# Autodesk Inventor assembly: The Real Chassis
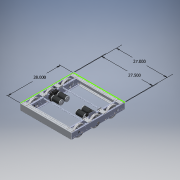
[picture p0: Inventor's stored thumbnail of the model, 180x180]
Saved by Autodesk Inventor 2018 (Build 220112000, 112)
## iProperties
Created: 2015-12-07
Part Number: The Real Chassis
Description: STEP AP214
Document SubType Name: Assembly
Designer: 20dbrownell
Sending System: SolidWorks 2014
Preprocessor: SwSTEP 2.0
Title: AM14U3 Square REV1-1.STEP
Revision Number: ANY
## Documents named in this file (3)
- C:\Users\20dbrownell\Documents\GitHub\RobotDesigns2018\The Real Chassis.iam
- C:\Users\20dbrownell\Downloads\AM14U3 Square Half.iam
- H:\Robotics\am-0255+2.5inch+CIM+Motor.ipt
## Components (10 placed, 3 different names)
1. AM14U3 Square Half_1 [sub-assembly] — Mate:1, Mate:2, Mate:5, Mate:6, Mate:9, Mate:10, Mate:14, Mate:16
2. AM14U3 Square Half_2 [sub-assembly] — Mate:3, Mate:4, Mate:7, Mate:8, Mate:11, Mate:12, Mate:13, Mate:15
3. am-0255+2.5inch+CIM+Motor:1 — Mate:4, Mate:7
4. am-0255+2.5inch+CIM+Motor:2 — Mate:3, Mate:8
5. am-0255+2.5inch+CIM+Motor:3 — Mate:2, Mate:6
6. am-0255+2.5inch+CIM+Motor:4 — Mate:1, Mate:5
7. am-0255+2.5inch+CIM+Motor:5 — Mate:10, Mate:16
8. am-0255+2.5inch+CIM+Motor:6 — Mate:11, Mate:15
9. am-0255+2.5inch+CIM+Motor:7 — Mate:12, Mate:13
10. am-0255+2.5inch+CIM+Motor:8 — Mate:9, Mate:14
## Relationships (16: Mate 16)
- Mate:1: AM14U3 Square Half_1 ↔ am-0255+2.5inch+CIM+Motor:4
- Mate:2: AM14U3 Square Half_1 ↔ am-0255+2.5inch+CIM+Motor:3
- Mate:3: AM14U3 Square Half_2 ↔ am-0255+2.5inch+CIM+Motor:2
- Mate:4: AM14U3 Square Half_2 ↔ am-0255+2.5inch+CIM+Motor:1
- Mate:5: AM14U3 Square Half_1 ↔ am-0255+2.5inch+CIM+Motor:4
- Mate:6: AM14U3 Square Half_1 ↔ am-0255+2.5inch+CIM+Motor:3
- Mate:7: AM14U3 Square Half_2 ↔ am-0255+2.5inch+CIM+Motor:1
- Mate:8: AM14U3 Square Half_2 ↔ am-0255+2.5inch+CIM+Motor:2
- Mate:9: AM14U3 Square Half_1 ↔ am-0255+2.5inch+CIM+Motor:8
- Mate:10: AM14U3 Square Half_1 ↔ am-0255+2.5inch+CIM+Motor:5
- Mate:11: AM14U3 Square Half_2 ↔ am-0255+2.5inch+CIM+Motor:6
- Mate:12: AM14U3 Square Half_2 ↔ am-0255+2.5inch+CIM+Motor:7
- Mate:13: AM14U3 Square Half_2 ↔ am-0255+2.5inch+CIM+Motor:7
- Mate:14: AM14U3 Square Half_1 ↔ am-0255+2.5inch+CIM+Motor:8
- Mate:15: AM14U3 Square Half_2 ↔ am-0255+2.5inch+CIM+Motor:6
- Mate:16: AM14U3 Square Half_1 ↔ am-0255+2.5inch+CIM+Motor:5
